# Autodesk Inventor assembly: sail2
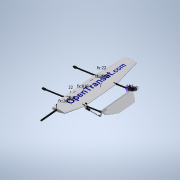
[picture p0: Inventor's stored thumbnail of the model, 180x180]
Saved by Autodesk Inventor 2020 (Build 240168000, 168)
## iProperties
Created: 2016-11-10
Part Number: sail2
Document SubType Name: Assembly
Designer: jous
Mass: 12117.7 g
Surface Area: 11891.4 cm^2
Volume: 12117.7 cm^3
Density: 1 g/cm^3
Author: jous
## Documents named in this file (18)
- C:\Users\jous\Desktop\boat\sail.iam
- C:\Users\jous\Desktop\boat\H4FM_0608_08.ipt
- C:\Users\jous\Desktop\boat\washer3.ipt
- C:\Users\jous\Desktop\boat\H4FM_0405_04.ipt
- C:\Users\jous\Desktop\boat\sail_skeleton.ipt
- C:\Users\jous\Desktop\boat\tail.ipt
- C:\Users\jous\Desktop\boat\sail.ipt
- C:\Users\jous\Desktop\boat\actuator_bracket1.ipt
- C:\Users\jous\Desktop\boat\actuator_shaft.ipt
- C:\Users\jous\Desktop\boat\actuator_bracket2.ipt
- C:\Users\jous\Desktop\boat\actuator\Firgelli L16 50mm body(50).ipt
- C:\Users\jous\Desktop\boat\actuator\Firgelli L16 50mm as(Short).ipt
- C:\Users\jous\Desktop\boat\actuator_shaft2.ipt
- C:\Users\jous\Desktop\boat\actuator_bracket3.ipt
- C:\Users\jous\Desktop\boat\actuator_counterweight.ipt
- C:\Users\jous\Desktop\boat\sail_weight.ipt
- C:\Users\jous\Desktop\boat\tail_encoder_magnet.ipt
- C:\Users\jous\Desktop\boat\tail_encoder.ipt
## Components (25 placed, 17 different names)
1. sail_skeleton:1 — Angle:5, Rigid:1, Rigid:2, Rigid:4, Rotational:30, Rigid:5, tail angle, Rigid:44, Rigid:45, Rigid:47, Angle:7
2. sail:1 — Angle:5, Rotational:30
3. tail:1 — Rotational:24, Rotational:25, Mate:1, Mate:3, tail angle, Mate:4, Mate:5, Mate:7, Mate:8
4. washer3:3 — Rotational:24, Rotational:26
5. washer3:4 — Rotational:25
6. H4FM_0608_08:3 — Rigid:1, Rotational:26
7. H4FM_0608_08:4 — Rigid:2
8. washer3:5 — Rotational:41, Rotational:42
9. washer3:6 — Rigid:4
10. actuator_bracket1:1 — Rigid:5, Rotational:35, Rotational:38, Rotational:39
11. actuator_shaft:1 — Rigid:46
12. actuator_bracket2:1 — Mate:1, Mate:3, Cylindrical:37, Rotational:36, Rotational:40, Mate:7
13. Firgelli L16 50mm body(50):1 — Rotational:35, Cylindrical:38
14. Firgelli L16 50mm as(Short):1 — Cylindrical:37, Cylindrical:38
15. actuator_shaft2:1 — Rotational:36
16. H4FM_0405_04:7 — Rotational:38, Rigid:46
17. H4FM_0405_04:8 — Rotational:39
18. H4FM_0405_04:9 — Rotational:40
19. actuator_bracket3:1 — Mate:4, Mate:5, Mate:8
20. actuator_counterweight:1
21. sail_weight:1 — Rigid:44
22. sail_weight:2 — Rigid:45
23. H4FM_0608_08:5 — Rigid:47, Rotational:41
24. tail_encoder_magnet:1 — Rotational:42, Rotational:43
25. tail_encoder:1 — Rotational:43, Angle:7
## Relationships (31: RevoluteJoint 12, WeldJoint 8, Mate 6, Angle 3, CylindricalJoint 2)
- Angle:5 (180 deg): sail_skeleton:1 ↔ sail:1
- Rotational:24 [RevoluteJoint]: tail:1 ↔ washer3:3
- Rotational:25 [RevoluteJoint]: tail:1 ↔ washer3:4
- Rigid:1 [WeldJoint]: sail_skeleton:1 ↔ H4FM_0608_08:3
- Rigid:2 [WeldJoint]: sail_skeleton:1 ↔ H4FM_0608_08:4
- Rotational:26 [RevoluteJoint]: washer3:3 ↔ H4FM_0608_08:3
- Rigid:4 [WeldJoint]: sail_skeleton:1 ↔ washer3:6
- Rotational:30 [RevoluteJoint] (-10 mm): sail_skeleton:1 ↔ sail:1
- Rigid:5 [WeldJoint]: sail_skeleton:1 ↔ actuator_bracket1:1
- Mate:1: tail:1 ↔ actuator_bracket2:1
- Mate:3: tail:1 ↔ actuator_bracket2:1
- tail angle [Angle] (-25 deg): sail_skeleton:1 ↔ tail:1
- Rotational:35 [RevoluteJoint] (12 mm): actuator_bracket1:1 ↔ Firgelli L16 50mm body(50):1
- Cylindrical:37: actuator_bracket2:1 ↔ Firgelli L16 50mm as(Short):1
- Cylindrical:38: Firgelli L16 50mm body(50):1 ↔ Firgelli L16 50mm as(Short):1
- Rotational:36 [RevoluteJoint] (-5 mm): actuator_bracket2:1 ↔ actuator_shaft2:1
- Rotational:38 [RevoluteJoint]: actuator_bracket1:1 ↔ H4FM_0405_04:7
- Rotational:39 [RevoluteJoint]: actuator_bracket1:1 ↔ H4FM_0405_04:8
- Rotational:40 [RevoluteJoint]: actuator_bracket2:1 ↔ H4FM_0405_04:9
- Mate:4: tail:1 ↔ actuator_bracket3:1
- Mate:5: tail:1 ↔ actuator_bracket3:1
- Rigid:44 [WeldJoint]: sail_skeleton:1 ↔ sail_weight:1
- Rigid:45 [WeldJoint]: sail_skeleton:1 ↔ sail_weight:2
- Rigid:46 [WeldJoint] (-3 mm): actuator_shaft:1 ↔ H4FM_0405_04:7
- Mate:7 (-3 mm): tail:1 ↔ actuator_bracket2:1
- Mate:8 (3 mm): tail:1 ↔ actuator_bracket3:1
- Rigid:47 [WeldJoint]: sail_skeleton:1 ↔ H4FM_0608_08:5
- Rotational:41 [RevoluteJoint]: washer3:5 ↔ H4FM_0608_08:5
- Rotational:42 [RevoluteJoint]: washer3:5 ↔ tail_encoder_magnet:1
- Rotational:43 [RevoluteJoint] (3.61 mm): tail_encoder_magnet:1 ↔ tail_encoder:1
- Angle:7 (0 deg): sail_skeleton:1 ↔ tail_encoder:1
## Named parameters: sail_height = 1300 mm, tail_offset = 260 mm, PCB_thickness = 1.65 mm, wall = 3 mm, PCB_height = 3.46 mm
